# Autodesk Inventor assembly: VER2.0
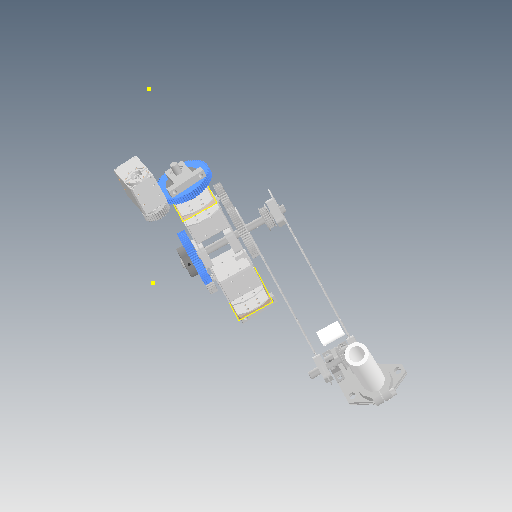
[picture p0: Inventor's stored thumbnail of the model, 512x512]
Saved by Autodesk Inventor 2020.5 (Build 245400000, 400)
## iProperties
Created: 2022-10-31
Part Number: VER2.0
Document SubType Name: Assembly
Designer: Administrator
Author: Administrator
## Documents named in this file (24)
- C:\Users\Administrator\Documents\kamuy2\kamuy2\VER2.0.iam
- C:\Users\Administrator\Documents\kamuy2\kamuy2\Parts\x-540_idle.ipt
- C:\Users\Administrator\Documents\kamuy2\kamuy2\Parts\XW540.N105.I101.ipt
- C:\Users\Administrator\Documents\kamuy2\kamuy2\Parts\GEABP1.0-32-10-A-12-KFC22-K3_Autodesk_Inventor_2020_20221101\AIS2020\GEABP1_0-32-10-A-12-KFC22-K3.iam
- C:\Users\Administrator\Documents\kamuy2\kamuy2\Parts\Part2.ipt
- C:\Users\Administrator\Documents\kamuy2\kamuy2\Parts\GEYK1.0-70-10-B-10K_Autodesk_Inventor_2020_20221114\AIS2020\GEYK1_0-70-10-B-10K.iam
- C:\Users\Administrator\Documents\kamuy2\kamuy2\Parts\GEABP1.0-70-10-A-19-KFC30-K3_Autodesk_Inventor_2020_20221114\AIS2020\GEABP1_0-70-10-A-19-KFC30-K3.iam
- C:\Users\Administrator\Documents\kamuy2\kamuy2\Parts\PIJX30-20-150_Autodesk_Inventor_2020_20221115\PIJX30-20-150.ipt
- C:\Users\Administrator\Documents\kamuy2\kamuy2\Parts\C-SHA10_Autodesk_Inventor_2020_20221104\AIS2020\C-SHA10.iam
- C:\Users\Administrator\Documents\kamuy2\kamuy2\Part16.ipt
- C:\Users\Administrator\Documents\kamuy2\kamuy2\Parts\HTPA30S3M060-A-N10_Autodesk_Inventor_2020_20221115\AIS2020\HTPA30S3M060-A-N10.iam
- C:\Users\Administrator\Documents\kamuy2\kamuy2\Part1.ipt
- C:\Users\Administrator\Documents\kamuy2\kamuy2\Part13.ipt
- C:\Users\Administrator\Documents\kamuy2\kamuy2\Part17.ipt
- C:\Users\Administrator\Documents\kamuy2\kamuy2\Parts\SMYHF10_STEP_AP203AP214\SMYHF10_203.ipt
- C:\Users\Administrator\Documents\kamuy2\kamuy2\Parts\BGHK6800VV-30_Autodesk_Inventor_2020_20221102\AIS2020\BGHK6800VV-30.iam
- C:\Users\Administrator\Documents\kamuy2\kamuy2\Parts\NSFMKR10-67-KA22-A20_Autodesk_Inventor_2020_20221116\AIS2020\NSFMKR10-67-KA22-A20.iam
- C:\Users\Administrator\Documents\kamuy2\kamuy2\Parts\NSFMR10-37_Autodesk_Inventor_2020_20221116\AIS2020\NSFMR10-37(000_000).iam
- C:\Users\Administrator\Documents\kamuy2\kamuy2\Part20.ipt
- C:\Users\Administrator\Documents\kamuy2\kamuy2\Parts\SMYHF30_STEP_AP203AP214\SMYHF30_203.ipt
- C:\Users\Administrator\Documents\kamuy2\kamuy2\Part22.ipt
- C:\Users\Administrator\Documents\kamuy2\kamuy2\Parts\RORPOS20-L30_Autodesk_Inventor_2020_20221117\AIS2020\RORPOS20-L30.iam
- C:\Users\Administrator\Documents\kamuy2\kamuy2\Parts\NSFMRRA10-74-B3-S3-KC31.5-A11_Autodesk_Inventor_2020_20221116\AIS2020\NSFMRRA10-74-B3-S3-KC31_5-A11(000_000).iam
- C:\Users\Administrator\Documents\kamuy2\kamuy2\Parts\NSFMKRRA10-144-F3-S6-KA5-A18-KB108.5-B11_Autodesk_Inventor_2020_20221117\AIS2020\NSFMKRRA10-144-F3-S6-KA5-A18-KB108_5-B11.iam
## Components (39 placed, 23 different names)
1. Part2:1
2. x-540_idle:3 — フラッシュ:58, フラッシュ:66, フラッシュ:68, メイト:154, メイト:166, フラッシュ:103, メイト:256, フラッシュ:140, メイト:258
3. GEABP1_0-32-10-A-12-KFC22-K3:4 [sub-assembly] — フラッシュ:69
4. GEYK1_0-70-10-B-10K:2 [sub-assembly] — フラッシュ:61, メイト:248, フラッシュ:136
5. x-540_idle:4 — フラッシュ:58, メイト:85, メイト:86, フラッシュ:66, フラッシュ:68, フラッシュ:100, メイト:168, メイト:178, メイト:179, メイト:180, メイト:183
6. GEABP1_0-32-10-A-12-KFC22-K3:5 [sub-assembly] — メイト:85, メイト:86, フラッシュ:61
7. GEABP1_0-70-10-A-19-KFC30-K3:1 [sub-assembly] — フラッシュ:69, フラッシュ:123, メイト:255
8. PIJX30-20-150:1 — メイト:244, メイト:245
9. C-SHA10:1 [sub-assembly] — フラッシュ:89, メイト:235, フラッシュ:131, フラッシュ:133, メイト:249, メイト:264
10. C-SHA10:2 [sub-assembly] — フラッシュ:89, メイト:237, フラッシュ:131, メイト:250
11. Part16:1 — フラッシュ:96, フラッシュ:122, メイト:236
12. Part16:2 — フラッシュ:92, メイト:170, メイト:258
13. Part16:3 — フラッシュ:92, メイト:154, メイト:168, メイト:171, フラッシュ:141
14. Part16:4 — フラッシュ:96, メイト:164, メイト:219, メイト:230, メイト:266
15. Part16:5 — メイト:219, フラッシュ:122, メイト:234, メイト:252, フラッシュ:139
16. HTPA30S3M060-A-N10:1 [sub-assembly] — フラッシュ:138, メイト:263
17. HTPA30S3M060-A-N10:2 [sub-assembly] — メイト:164, フラッシュ:138, メイト:259
18. Part1:2 — フラッシュ:100, フラッシュ:101, メイト:171, フラッシュ:140, フラッシュ:141
19. Part1:3 — フラッシュ:101, メイト:166, メイト:170, メイト:183, メイト:257
20. Part13:1 — フラッシュ:103, メイト:172, フラッシュ:104, フラッシュ:108, メイト:208
21. Part17:1 — メイト:172, フラッシュ:104, メイト:174, フラッシュ:105, メイト:177, フラッシュ:108
22. SMYHF10_203:1 — メイト:174, フラッシュ:105, メイト:254
23. GEYK1_0-70-10-B-10K:4 [sub-assembly] — メイト:177, メイト:207, メイト:267
24. Part13:2 — メイト:178, メイト:179, メイト:180, メイト:194, フラッシュ:110, メイト:214
25. SMYHF10_203:2 — メイト:185, メイト:187, メイト:213
26. Part17:2 — メイト:185, メイト:187, メイト:194, フラッシュ:110, メイト:211, メイト:215
27. BGHK6800VV-30:3 [sub-assembly] — メイト:205, メイト:209, フラッシュ:115, フラッシュ:116, フラッシュ:144, フラッシュ:145, メイト:267
28. GEABP1_0-32-10-A-12-KFC22-K3:8 [sub-assembly] — メイト:203, メイト:204
29. XW540.N105.I101:5 — メイト:203, メイト:204, メイト:205, フラッシュ:144, フラッシュ:145
30. NSFMKR10-67-KA22-A20:1 [sub-assembly] — メイト:207, メイト:208, メイト:209, メイト:254
31. BGHK6800VV-30:4 [sub-assembly] — フラッシュ:115, フラッシュ:116, メイト:211, メイト:212
32. NSFMR10-37(000_000):1 [sub-assembly] — メイト:212, メイト:213, メイト:214, メイト:215
33. Part20:1 — フラッシュ:123, メイト:236, メイト:237, メイト:261, フラッシュ:142, メイト:265
34. Part20:2 — メイト:230, メイト:234, メイト:235, メイト:247, フラッシュ:137, メイト:251, メイト:253, フラッシュ:142, メイト:265
35. SMYHF30_203:1 — メイト:242, メイト:244, フラッシュ:135, メイト:246
36. Part22:1 — フラッシュ:133, メイト:242, メイト:245, フラッシュ:135, メイト:246, メイト:249, メイト:250
37. RORPOS20-L30:1 [sub-assembly] — メイト:247, メイト:251
38. NSFMRRA10-74-B3-S3-KC31_5-A11(000_000):1 [sub-assembly] — メイト:252, フラッシュ:139, メイト:253, メイト:263, メイト:264
39. NSFMKRRA10-144-F3-S6-KA5-A18-KB108_5-B11:1 [sub-assembly] — メイト:248, フラッシュ:136, フラッシュ:137, メイト:255, メイト:256, メイト:257, メイト:259, メイト:261, メイト:266
## Relationships (91: Mate 60, Flush 31)
- [Mate] (4 mm): x-540_idle:3 ↔ GEABP1_0-32-10-A-12-KFC22-K3:4
- [Mate]: x-540_idle:3 ↔ GEABP1_0-32-10-A-12-KFC22-K3:4
- フラッシュ:58 [Flush]: x-540_idle:3 ↔ x-540_idle:4
- メイト:85 [Mate]: x-540_idle:4 ↔ GEABP1_0-32-10-A-12-KFC22-K3:5
- メイト:86 [Mate] (4 mm): x-540_idle:4 ↔ GEABP1_0-32-10-A-12-KFC22-K3:5
- フラッシュ:61 [Flush]: GEYK1_0-70-10-B-10K:2 ↔ GEABP1_0-32-10-A-12-KFC22-K3:5
- フラッシュ:66 [Flush]: x-540_idle:3 ↔ x-540_idle:4
- フラッシュ:68 [Flush]: x-540_idle:3 ↔ x-540_idle:4
- フラッシュ:69 [Flush]: GEABP1_0-32-10-A-12-KFC22-K3:4 ↔ GEABP1_0-70-10-A-19-KFC30-K3:1
- フラッシュ:89 [Flush]: C-SHA10:1 ↔ C-SHA10:2
- フラッシュ:92 [Flush]: Part16:2 ↔ Part16:3
- メイト:154 [Mate] (15.591 mm): x-540_idle:3 ↔ Part16:3
- フラッシュ:96 [Flush]: Part16:1 ↔ Part16:4
- メイト:164 [Mate] (7 mm): Part16:4 ↔ HTPA30S3M060-A-N10:2
- フラッシュ:100 [Flush]: x-540_idle:4 ↔ Part1:2
- フラッシュ:101 [Flush]: Part1:2 ↔ Part1:3
- メイト:166 [Mate]: x-540_idle:3 ↔ Part1:3
- フラッシュ:103 [Flush]: x-540_idle:3 ↔ Part13:1
- メイト:168 [Mate] (15.591 mm): x-540_idle:4 ↔ Part16:3
- メイト:170 [Mate]: Part16:2 ↔ Part1:3
- メイト:171 [Mate]: Part16:3 ↔ Part1:2
- メイト:172 [Mate] (15 mm): Part13:1 ↔ Part17:1
- フラッシュ:104 [Flush]: Part13:1 ↔ Part17:1
- メイト:174 [Mate]: Part17:1 ↔ SMYHF10_203:1
- フラッシュ:105 [Flush] (0.1 mm): Part17:1 ↔ SMYHF10_203:1
- メイト:177 [Mate] (5 mm): Part17:1 ↔ GEYK1_0-70-10-B-10K:4
- メイト:178 [Mate]: x-540_idle:4 ↔ Part13:2
- メイト:179 [Mate]: x-540_idle:4 ↔ Part13:2
- メイト:180 [Mate]: x-540_idle:4 ↔ Part13:2
- メイト:183 [Mate]: x-540_idle:4 ↔ Part1:3
- メイト:185 [Mate]: SMYHF10_203:2 ↔ Part17:2
- メイト:187 [Mate]: SMYHF10_203:2 ↔ Part17:2
- メイト:194 [Mate] (15 mm): Part13:2 ↔ Part17:2
- フラッシュ:108 [Flush]: Part13:1 ↔ Part17:1
- フラッシュ:110 [Flush]: Part13:2 ↔ Part17:2
- メイト:203 [Mate]: GEABP1_0-32-10-A-12-KFC22-K3:8 ↔ XW540.N105.I101:5
- メイト:204 [Mate]: GEABP1_0-32-10-A-12-KFC22-K3:8 ↔ XW540.N105.I101:5
- メイト:205 [Mate] (6.591 mm): BGHK6800VV-30:3 ↔ XW540.N105.I101:5
- メイト:207 [Mate]: GEYK1_0-70-10-B-10K:4 ↔ NSFMKR10-67-KA22-A20:1
- メイト:208 [Mate]: Part13:1 ↔ NSFMKR10-67-KA22-A20:1
- メイト:209 [Mate]: BGHK6800VV-30:3 ↔ NSFMKR10-67-KA22-A20:1
- フラッシュ:115 [Flush]: BGHK6800VV-30:3 ↔ BGHK6800VV-30:4
- フラッシュ:116 [Flush]: BGHK6800VV-30:3 ↔ BGHK6800VV-30:4
- メイト:211 [Mate] (4 mm): Part17:2 ↔ BGHK6800VV-30:4
- メイト:212 [Mate]: BGHK6800VV-30:4 ↔ NSFMR10-37(000_000):1
- メイト:213 [Mate]: SMYHF10_203:2 ↔ NSFMR10-37(000_000):1
- メイト:214 [Mate]: Part13:2 ↔ NSFMR10-37(000_000):1
- メイト:215 [Mate]: Part17:2 ↔ NSFMR10-37(000_000):1
- メイト:219 [Mate] (168 mm): Part16:4 ↔ Part16:5
- フラッシュ:122 [Flush]: Part16:1 ↔ Part16:5
- フラッシュ:123 [Flush]: GEABP1_0-70-10-A-19-KFC30-K3:1 ↔ Part20:1
- メイト:230 [Mate]: Part16:4 ↔ Part20:2
- メイト:234 [Mate]: Part16:5 ↔ Part20:2
- メイト:235 [Mate] (6 mm): C-SHA10:1 ↔ Part20:2
- メイト:236 [Mate]: Part16:1 ↔ Part20:1
- メイト:237 [Mate] (6 mm): C-SHA10:2 ↔ Part20:1
- フラッシュ:131 [Flush]: C-SHA10:1 ↔ C-SHA10:2
- フラッシュ:133 [Flush]: C-SHA10:1 ↔ Part22:1
- メイト:242 [Mate]: SMYHF30_203:1 ↔ Part22:1
- メイト:244 [Mate]: PIJX30-20-150:1 ↔ SMYHF30_203:1
- メイト:245 [Mate]: PIJX30-20-150:1 ↔ Part22:1
- フラッシュ:135 [Flush]: SMYHF30_203:1 ↔ Part22:1
- メイト:246 [Mate]: SMYHF30_203:1 ↔ Part22:1
- メイト:247 [Mate] (2.5 mm): Part20:2 ↔ RORPOS20-L30:1
- メイト:248 [Mate]: GEYK1_0-70-10-B-10K:2 ↔ NSFMKRRA10-144-F3-S6-KA5-A18-KB108_5-B11:1
- フラッシュ:136 [Flush] (-3 mm): GEYK1_0-70-10-B-10K:2 ↔ NSFMKRRA10-144-F3-S6-KA5-A18-KB108_5-B11:1
- フラッシュ:137 [Flush] (6 mm): Part20:2 ↔ NSFMKRRA10-144-F3-S6-KA5-A18-KB108_5-B11:1
- フラッシュ:138 [Flush]: HTPA30S3M060-A-N10:1 ↔ HTPA30S3M060-A-N10:2
- メイト:249 [Mate]: C-SHA10:1 ↔ Part22:1
- メイト:250 [Mate]: C-SHA10:2 ↔ Part22:1
- メイト:251 [Mate]: Part20:2 ↔ RORPOS20-L30:1
- メイト:252 [Mate]: Part16:5 ↔ NSFMRRA10-74-B3-S3-KC31_5-A11(000_000):1
- フラッシュ:139 [Flush] (-3 mm): Part16:5 ↔ NSFMRRA10-74-B3-S3-KC31_5-A11(000_000):1
- メイト:253 [Mate]: Part20:2 ↔ NSFMRRA10-74-B3-S3-KC31_5-A11(000_000):1
- メイト:254 [Mate]: SMYHF10_203:1 ↔ NSFMKR10-67-KA22-A20:1
- メイト:255 [Mate]: GEABP1_0-70-10-A-19-KFC30-K3:1 ↔ NSFMKRRA10-144-F3-S6-KA5-A18-KB108_5-B11:1
- メイト:256 [Mate] (31.591 mm): x-540_idle:3 ↔ NSFMKRRA10-144-F3-S6-KA5-A18-KB108_5-B11:1
- メイト:257 [Mate] (-28.819 mm): Part1:3 ↔ NSFMKRRA10-144-F3-S6-KA5-A18-KB108_5-B11:1
- フラッシュ:140 [Flush]: x-540_idle:3 ↔ Part1:2
- メイト:258 [Mate] (15.591 mm): x-540_idle:3 ↔ Part16:2
- メイト:259 [Mate]: HTPA30S3M060-A-N10:2 ↔ NSFMKRRA10-144-F3-S6-KA5-A18-KB108_5-B11:1
- メイト:261 [Mate]: Part20:1 ↔ NSFMKRRA10-144-F3-S6-KA5-A18-KB108_5-B11:1
- メイト:263 [Mate]: HTPA30S3M060-A-N10:1 ↔ NSFMRRA10-74-B3-S3-KC31_5-A11(000_000):1
- メイト:264 [Mate]: C-SHA10:1 ↔ NSFMRRA10-74-B3-S3-KC31_5-A11(000_000):1
- フラッシュ:141 [Flush] (12.859 mm): Part16:3 ↔ Part1:2
- フラッシュ:142 [Flush]: Part20:1 ↔ Part20:2
- メイト:265 [Mate]: Part20:1 ↔ Part20:2
- メイト:266 [Mate]: Part16:4 ↔ NSFMKRRA10-144-F3-S6-KA5-A18-KB108_5-B11:1
- フラッシュ:144 [Flush]: BGHK6800VV-30:3 ↔ XW540.N105.I101:5
- フラッシュ:145 [Flush]: BGHK6800VV-30:3 ↔ XW540.N105.I101:5
- メイト:267 [Mate] (4 mm): GEYK1_0-70-10-B-10K:4 ↔ BGHK6800VV-30:3
## Named parameters: d99_d5 = 4 mm, d100_d6 = 0 mm
